# Autodesk Inventor assembly: STEFAN
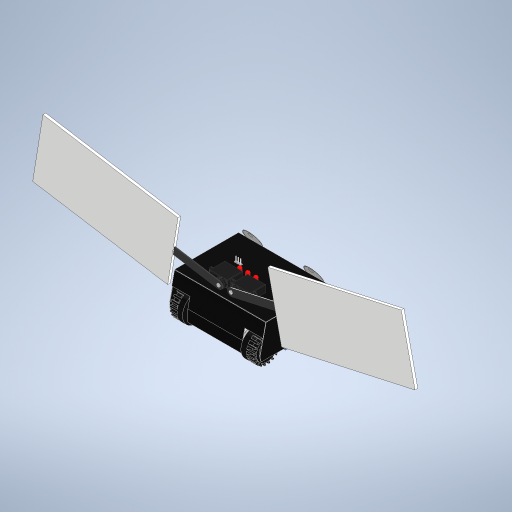
[picture p0: Inventor's stored thumbnail of the model, 512x512]
Saved by Autodesk Inventor 2023 (Build 270158000, 158)
## iProperties
Created: 2023-07-07
Part Number: STEFAN
Document SubType Name: Assembly
Designer: Kamil
Author: Kamil
## Documents named in this file (19)
- C:\Users\Kamil\Desktop\MojeRoboty\Stefan\mechanics 2\STEFAN.iam
- C:\Users\Kamil\Desktop\MojeRoboty\Stefan\mechanics 2\podstawa.ipt
- C:\Users\Kamil\Desktop\MojeRoboty\Stefan\mechanics 2\sciana_prawa_nowa.ipt
- C:\Users\Kamil\Desktop\MojeRoboty\Stefan\mechanics 2\n20 motor.ipt
- C:\Users\Kamil\Desktop\MojeRoboty\Stefan\mechanics 2\uchwyt_nowy.ipt
- C:\Users\Kamil\Desktop\MojeRoboty\Stefan\mechanics 2\koło_minisumo.ipt
- C:\Users\Kamil\Desktop\MojeRoboty\Stefan\mechanics 2\sciana_prawa_nowa_MIR.ipt
- C:\Users\Kamil\Desktop\MojeRoboty\Stefan\mechanics 2\plytka_dol.iam
- C:\Users\Kamil\Desktop\MojeRoboty\Stefan\mechanics 2\plug_nowy.ipt
- C:\Users\Kamil\Desktop\MojeRoboty\Stefan\mechanics 2\GP2Y0A41SK0F.ipt
- C:\Users\Kamil\Desktop\MojeRoboty\Stefan\mechanics 2\dach.ipt
- C:\Users\Kamil\Desktop\MojeRoboty\Stefan\mechanics 2\tyl.ipt
- C:\Users\Kamil\Desktop\MojeRoboty\Stefan\mechanics 2\servo_mini_1370hd_cos.ipt
- C:\Users\Kamil\Desktop\MojeRoboty\Stefan\mechanics 2\pokrywa lewa.ipt
- C:\Users\Kamil\Desktop\MojeRoboty\Stefan\mechanics 2\pokrywa prawa.ipt
- C:\Users\Kamil\Desktop\MojeRoboty\Stefan\mechanics 2\plytka_gora.iam
- C:\Users\Kamil\Desktop\MojeRoboty\Stefan\mechanics 2\oko.ipt
- C:\Users\Kamil\Desktop\MojeRoboty\Stefan\mechanics 2\buzia.ipt
- C:\Users\Kamil\Desktop\MojeRoboty\Stefan\mechanics 2\reka.ipt
## Components (24 placed, 18 different names)
1. podstawa:1 — Równoległe:1, Zestawiające:1, Zestawiające:2, Zestawiające:7, Równoległe:4, Równoległe:5, Równoległe:6, Zestawiające:12, Zestawiające:13, Równoległe:7, Równoległe:10, Równoległe:11, Równoległe:14, Zestawiające:28, Zestawiające:31
2. sciana_prawa_nowa:1 — Równoległe:1, Zestawiające:1, Zestawiające:2, Zestawiające:14, Zestawiające:16, Zestawiające:20, Zestawiające:30
3. n20 motor:1 — Zestawiające:5, Zestawiające:6, Równoległe:3, Równoległe:4, Zestawiające:8, Zestawiające:9
4. n20 motor:2 — Zestawiające:3, Zestawiające:4, Równoległe:2, Zestawiające:10, Zestawiające:11
5. uchwyt_nowy:1 — Zestawiające:3, Zestawiające:4, Równoległe:2, Zestawiające:5, Zestawiające:6, Równoległe:3, Zestawiające:7, Równoległe:5
6. koło_minisumo:1 — Zestawiające:8, Zestawiające:9
7. koło_minisumo:2 — Zestawiające:10, Zestawiające:11
8. sciana_prawa_nowa_MIR:1 — Równoległe:6, Zestawiające:12, Zestawiające:13, Zestawiające:15, Zestawiające:17, Zestawiające:22, Zestawiające:23, Zestawiające:27, Równoległe:15
9. plytka_dol:1 [sub-assembly] — Zestawiające:14, Zestawiające:15, Zestawiające:16, Równoległe:16
10. plug_nowy:1 — Zestawiające:17, Równoległe:7, Zestawiające:18, Zestawiające:19, Zestawiające:21, Zestawiające:33, Zestawiające:34, Równoległe:17
11. GP2Y0A41SK0F:1 — Zestawiające:18, Równoległe:8, Równoległe:9
12. GP2Y0A41SK0F:2 — Zestawiające:19, Równoległe:8, Równoległe:9
13. dach:1 — Zestawiające:20, Równoległe:10, Zestawiające:21, Zestawiające:24, Zestawiające:25, Równoległe:13
14. tyl:1 — Zestawiające:22, Równoległe:11, Zestawiające:23, Zestawiające:29, Zestawiające:32
15. servo_mini_1370hd_cos:1 — Zestawiające:25, Zestawiające:26, Równoległe:12, Równoległe:13, Zestawiające:35, Zestawiające:36
16. servo_mini_1370hd_cos:2 — Zestawiające:24, Zestawiające:26, Równoległe:12, Równoległe:14, Zestawiające:37, Zestawiające:38
17. pokrywa lewa:1 — Zestawiające:27, Zestawiające:28, Zestawiające:29
18. pokrywa prawa:1 — Zestawiające:30, Zestawiające:31, Zestawiające:32
19. plytka_gora:1 [sub-assembly] — Równoległe:15, Równoległe:16
20. oko:1 — Zestawiające:33
21. oko:2 — Zestawiające:34
22. buzia:1 — Równoległe:17
23. reka:1 — Zestawiające:35, Zestawiające:36
24. reka:2 — Zestawiające:37, Zestawiające:38
## Relationships (55: Mate 38, Flush 17)
- Równoległe:1 [Flush] (0.6 mm): podstawa:1 ↔ sciana_prawa_nowa:1
- Zestawiające:1 [Mate]: podstawa:1 ↔ sciana_prawa_nowa:1
- Zestawiające:2 [Mate]: podstawa:1 ↔ sciana_prawa_nowa:1
- Zestawiające:3 [Mate]: n20 motor:2 ↔ uchwyt_nowy:1
- Zestawiające:4 [Mate]: n20 motor:2 ↔ uchwyt_nowy:1
- Równoległe:2 [Flush]: n20 motor:2 ↔ uchwyt_nowy:1
- Zestawiające:5 [Mate]: n20 motor:1 ↔ uchwyt_nowy:1
- Zestawiające:6 [Mate]: n20 motor:1 ↔ uchwyt_nowy:1
- Równoległe:3 [Flush]: n20 motor:1 ↔ uchwyt_nowy:1
- Zestawiające:7 [Mate]: podstawa:1 ↔ uchwyt_nowy:1
- Równoległe:4 [Flush]: podstawa:1 ↔ n20 motor:1
- Równoległe:5 [Flush]: podstawa:1 ↔ uchwyt_nowy:1
- Zestawiające:8 [Mate]: n20 motor:1 ↔ koło_minisumo:1
- Zestawiające:9 [Mate] (2 mm): n20 motor:1 ↔ koło_minisumo:1
- Zestawiające:10 [Mate] (2 mm): n20 motor:2 ↔ koło_minisumo:2
- Zestawiające:11 [Mate]: n20 motor:2 ↔ koło_minisumo:2
- Równoległe:6 [Flush] (-0.6 mm): podstawa:1 ↔ sciana_prawa_nowa_MIR:1
- Zestawiające:12 [Mate]: podstawa:1 ↔ sciana_prawa_nowa_MIR:1
- Zestawiające:13 [Mate]: podstawa:1 ↔ sciana_prawa_nowa_MIR:1
- Zestawiające:14 [Mate]: sciana_prawa_nowa:1 ↔ plytka_dol:1
- Zestawiające:15 [Mate]: sciana_prawa_nowa_MIR:1 ↔ plytka_dol:1
- Zestawiające:16 [Mate]: sciana_prawa_nowa:1 ↔ plytka_dol:1
- Zestawiające:17 [Mate]: sciana_prawa_nowa_MIR:1 ↔ plug_nowy:1
- Równoległe:7 [Flush]: podstawa:1 ↔ plug_nowy:1
- Zestawiające:18 [Mate]: plug_nowy:1 ↔ GP2Y0A41SK0F:1
- Zestawiające:19 [Mate]: plug_nowy:1 ↔ GP2Y0A41SK0F:2
- Równoległe:8 [Flush]: GP2Y0A41SK0F:1 ↔ GP2Y0A41SK0F:2
- Równoległe:9 [Flush]: GP2Y0A41SK0F:1 ↔ GP2Y0A41SK0F:2
- Zestawiające:20 [Mate]: sciana_prawa_nowa:1 ↔ dach:1
- Równoległe:10 [Flush]: podstawa:1 ↔ dach:1
- Zestawiające:21 [Mate]: plug_nowy:1 ↔ dach:1
- Zestawiające:22 [Mate]: sciana_prawa_nowa_MIR:1 ↔ tyl:1
- Równoległe:11 [Flush]: podstawa:1 ↔ tyl:1
- Zestawiające:23 [Mate] (0.74 mm): sciana_prawa_nowa_MIR:1 ↔ tyl:1
- Zestawiające:24 [Mate]: dach:1 ↔ servo_mini_1370hd_cos:2
- Zestawiające:25 [Mate]: dach:1 ↔ servo_mini_1370hd_cos:1
- Zestawiające:26 [Mate] (5 mm): servo_mini_1370hd_cos:1 ↔ servo_mini_1370hd_cos:2
- Równoległe:12 [Flush]: servo_mini_1370hd_cos:1 ↔ servo_mini_1370hd_cos:2
- Równoległe:13 [Flush] (10 mm): dach:1 ↔ servo_mini_1370hd_cos:1
- Równoległe:14 [Flush] (27.5 mm): podstawa:1 ↔ servo_mini_1370hd_cos:2
- Zestawiające:27 [Mate]: sciana_prawa_nowa_MIR:1 ↔ pokrywa lewa:1
- Zestawiające:28 [Mate]: podstawa:1 ↔ pokrywa lewa:1
- Zestawiające:29 [Mate]: tyl:1 ↔ pokrywa lewa:1
- Zestawiające:30 [Mate]: sciana_prawa_nowa:1 ↔ pokrywa prawa:1
- Zestawiające:31 [Mate]: podstawa:1 ↔ pokrywa prawa:1
- Zestawiające:32 [Mate]: tyl:1 ↔ pokrywa prawa:1
- Równoległe:15 [Flush] (2 mm): sciana_prawa_nowa_MIR:1 ↔ plytka_gora:1
- Równoległe:16 [Flush]: plytka_dol:1 ↔ plytka_gora:1
- Zestawiające:33 [Mate] (1 mm): plug_nowy:1 ↔ oko:1
- Zestawiające:34 [Mate] (1 mm): plug_nowy:1 ↔ oko:2
- Równoległe:17 [Flush]: plug_nowy:1 ↔ buzia:1
- Zestawiające:35 [Mate] (1 mm): servo_mini_1370hd_cos:1 ↔ reka:1
- Zestawiające:36 [Mate]: servo_mini_1370hd_cos:1 ↔ reka:1
- Zestawiające:37 [Mate] (1 mm): servo_mini_1370hd_cos:2 ↔ reka:2
- Zestawiające:38 [Mate]: servo_mini_1370hd_cos:2 ↔ reka:2
